# Autodesk Inventor assembly: PC104 Stack Ultra Low Profile
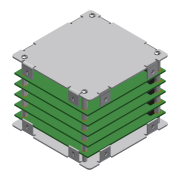
[picture p0: Inventor's stored thumbnail of the model, 180x180]
Saved by Autodesk Inventor 2018 (Build 220112000, 112)
## iProperties
Created: 2018-12-12
Part Number: PC104 Stack Ultra Low Profile
Document SubType Name: Assembly
Designer: R.P.SMITH
Mass: 216.229 g
Surface Area: 1807.71 cm^2
Volume: 132.857 cm^3
Density: 1.62753 g/cm^3
Author: R.P.SMITH
## Documents named in this file (10)
- D:\Documents\College\Semesters\4 - Fall\Senior Project 2\CADD Files\PC104 STACK ULTRA LOW PROFILE.iam
- D:\Documents\College\Semesters\4 - Fall\Senior Project 2\CADD Files\McMaster\93505A925_ALUM MALE-FEM THRDED HEX STANDOFF.ipt
- D:\Documents\College\Semesters\4 - Fall\Senior Project 2\CADD Files\Custom Parts\END MOUNT PC104 TOP.iam
- D:\Documents\College\Semesters\4 - Fall\Senior Project 2\CADD Files\McMaster\91772A106_18-8 SS PAN HEAD PHILLIPS MACHINE SCREW.ipt
- D:\Documents\College\Semesters\4 - Fall\Senior Project 2\CADD Files\Custom Parts\END MOUNT PC104 BOTTOM.iam
- D:\Documents\College\Semesters\4 - Fall\Senior Project 2\CADD Files\PC104 ISA BOARD VERY LOW PROFILE.iam
- D:\Documents\College\Semesters\4 - Fall\Senior Project 2\CADD Files\McMaster\93505A102_ALUM MALE-FEM THRDED HEX STANDOFF.ipt
- D:\Documents\College\Semesters\4 - Fall\Senior Project 2\CADD Files\McMaster\92510A696_ALUM UNTHRD SPACER.ipt
- D:\Documents\College\Semesters\4 - Fall\Senior Project 2\CADD Files\McMaster\91780A529_ALUM FEM THRDED HEX STANDOFF.ipt
- D:\Documents\College\Semesters\4 - Fall\Senior Project 2\CADD Files\McMaster\91772A112_18-8 SS PAN HEAD PHILLIPS MACHINE SCREW.ipt
## Components (39 placed, 9 different names)
1. 91772A106_18-8 SS PAN HEAD PHILLIPS MACHINE SCREW:1 — Insert:33
2. 91772A106_18-8 SS PAN HEAD PHILLIPS MACHINE SCREW:2 — Insert:34
3. 91772A106_18-8 SS PAN HEAD PHILLIPS MACHINE SCREW:3 — Insert:32
4. 91772A106_18-8 SS PAN HEAD PHILLIPS MACHINE SCREW:4 — Insert:31
5. END MOUNT PC104 TOP:2 [sub-assembly] — Insert:31, Insert:32, Insert:33, Insert:34, Insert:35, Insert:36, Insert:37, Insert:38
6. 93505A925_ALUM MALE-FEM THRDED HEX STANDOFF:1 — Insert:35, Insert:40
7. 93505A925_ALUM MALE-FEM THRDED HEX STANDOFF:2 — Insert:36
8. 93505A925_ALUM MALE-FEM THRDED HEX STANDOFF:3 — Insert:38, Insert:39
9. 93505A925_ALUM MALE-FEM THRDED HEX STANDOFF:4 — Insert:37
10. PC104 ISA BOARD VERY LOW PROFILE:4 [sub-assembly] — Insert:39, Insert:40, Mate:16, Insert:41, Insert:42, Insert:43, Insert:44
11. 93505A102_ALUM MALE-FEM THRDED HEX STANDOFF:1 — Insert:41
12. 93505A102_ALUM MALE-FEM THRDED HEX STANDOFF:2 — Insert:42
13. 93505A102_ALUM MALE-FEM THRDED HEX STANDOFF:3 — Insert:43
14. 93505A102_ALUM MALE-FEM THRDED HEX STANDOFF:4 — Insert:44
15. PC104 ISA BOARD VERY LOW PROFILE:3 [sub-assembly] — Mate:16, Mate:17, Insert:45, Insert:46, Insert:47, Insert:48
16. 93505A102_ALUM MALE-FEM THRDED HEX STANDOFF:5 — Insert:48
17. 93505A102_ALUM MALE-FEM THRDED HEX STANDOFF:12 — Insert:46
18. 93505A102_ALUM MALE-FEM THRDED HEX STANDOFF:14 — Insert:47
19. 93505A102_ALUM MALE-FEM THRDED HEX STANDOFF:13 — Insert:45
20. PC104 ISA BOARD VERY LOW PROFILE:2 [sub-assembly] — Mate:17, Mate:18, Insert:49, Insert:50, Insert:51, Insert:52
21. 93505A102_ALUM MALE-FEM THRDED HEX STANDOFF:6 — Insert:52
22. 93505A102_ALUM MALE-FEM THRDED HEX STANDOFF:9 — Insert:50
23. 93505A102_ALUM MALE-FEM THRDED HEX STANDOFF:10 — Insert:49
24. 93505A102_ALUM MALE-FEM THRDED HEX STANDOFF:11 — Insert:51
25. PC104 ISA BOARD VERY LOW PROFILE:1 [sub-assembly] — Mate:18, Mate:19, Insert:63, Insert:64, Insert:65, Insert:66
26. 91780A529_ALUM FEM THRDED HEX STANDOFF:1 — Insert:63
27. 91780A529_ALUM FEM THRDED HEX STANDOFF:2 — Insert:64
28. 91780A529_ALUM FEM THRDED HEX STANDOFF:3 — Insert:65
29. 91780A529_ALUM FEM THRDED HEX STANDOFF:4 — Insert:66
30. PC104 ISA BOARD VERY LOW PROFILE:5 [sub-assembly] — Mate:19, Mate:20, Insert:57, Insert:59, Insert:61, Insert:62
31. 92510A696_ALUM UNTHRD SPACER:1 — Insert:62
32. 92510A696_ALUM UNTHRD SPACER:2 — Insert:57, Insert:58
33. 92510A696_ALUM UNTHRD SPACER:3 — Insert:61
34. 92510A696_ALUM UNTHRD SPACER:4 — Insert:59, Insert:60
35. END MOUNT PC104 BOTTOM:1 [sub-assembly] — Mate:20, Insert:58, Insert:60, Insert:67, Insert:68, Insert:69, Insert:70
36. 91772A112_18-8 SS PAN HEAD PHILLIPS MACHINE SCREW:1 — Insert:67
37. 91772A112_18-8 SS PAN HEAD PHILLIPS MACHINE SCREW:2 — Insert:68
38. 91772A112_18-8 SS PAN HEAD PHILLIPS MACHINE SCREW:3 — Insert:70
39. 91772A112_18-8 SS PAN HEAD PHILLIPS MACHINE SCREW:4 — Insert:69
## Relationships (49: Insert 36, Mate 13)
- [Mate]: PC104 ISA BOARD VERY LOW PROFILE:2 ↔ PC104 ISA BOARD VERY LOW PROFILE:1
- [Mate]: PC104 ISA BOARD VERY LOW PROFILE:2 ↔ PC104 ISA BOARD VERY LOW PROFILE:1
- [Mate]: PC104 ISA BOARD VERY LOW PROFILE:3 ↔ PC104 ISA BOARD VERY LOW PROFILE:2
- [Mate]: PC104 ISA BOARD VERY LOW PROFILE:3 ↔ PC104 ISA BOARD VERY LOW PROFILE:2
- [Mate]: PC104 ISA BOARD VERY LOW PROFILE:4 ↔ PC104 ISA BOARD VERY LOW PROFILE:3
- [Mate]: PC104 ISA BOARD VERY LOW PROFILE:4 ↔ PC104 ISA BOARD VERY LOW PROFILE:3
- [Mate]: PC104 ISA BOARD VERY LOW PROFILE:1 ↔ PC104 ISA BOARD VERY LOW PROFILE:5
- [Mate]: PC104 ISA BOARD VERY LOW PROFILE:1 ↔ PC104 ISA BOARD VERY LOW PROFILE:5
- Insert:31: 91772A106_18-8 SS PAN HEAD PHILLIPS MACHINE SCREW:4 ↔ END MOUNT PC104 TOP:2
- Insert:32: 91772A106_18-8 SS PAN HEAD PHILLIPS MACHINE SCREW:3 ↔ END MOUNT PC104 TOP:2
- Insert:33: 91772A106_18-8 SS PAN HEAD PHILLIPS MACHINE SCREW:1 ↔ END MOUNT PC104 TOP:2
- Insert:34: 91772A106_18-8 SS PAN HEAD PHILLIPS MACHINE SCREW:2 ↔ END MOUNT PC104 TOP:2
- Insert:35: END MOUNT PC104 TOP:2 ↔ 93505A925_ALUM MALE-FEM THRDED HEX STANDOFF:1
- Insert:36: END MOUNT PC104 TOP:2 ↔ 93505A925_ALUM MALE-FEM THRDED HEX STANDOFF:2
- Insert:37: END MOUNT PC104 TOP:2 ↔ 93505A925_ALUM MALE-FEM THRDED HEX STANDOFF:4
- Insert:38: END MOUNT PC104 TOP:2 ↔ 93505A925_ALUM MALE-FEM THRDED HEX STANDOFF:3
- Insert:39: 93505A925_ALUM MALE-FEM THRDED HEX STANDOFF:3 ↔ PC104 ISA BOARD VERY LOW PROFILE:4
- Insert:40: 93505A925_ALUM MALE-FEM THRDED HEX STANDOFF:1 ↔ PC104 ISA BOARD VERY LOW PROFILE:4
- Mate:16 (9.525 mm): PC104 ISA BOARD VERY LOW PROFILE:4 ↔ PC104 ISA BOARD VERY LOW PROFILE:3
- Mate:17 (9.525 mm): PC104 ISA BOARD VERY LOW PROFILE:3 ↔ PC104 ISA BOARD VERY LOW PROFILE:2
- Mate:18 (9.525 mm): PC104 ISA BOARD VERY LOW PROFILE:2 ↔ PC104 ISA BOARD VERY LOW PROFILE:1
- Mate:19 (9.525 mm): PC104 ISA BOARD VERY LOW PROFILE:1 ↔ PC104 ISA BOARD VERY LOW PROFILE:5
- Insert:41: PC104 ISA BOARD VERY LOW PROFILE:4 ↔ 93505A102_ALUM MALE-FEM THRDED HEX STANDOFF:1
- Insert:42: PC104 ISA BOARD VERY LOW PROFILE:4 ↔ 93505A102_ALUM MALE-FEM THRDED HEX STANDOFF:2
- Insert:43: PC104 ISA BOARD VERY LOW PROFILE:4 ↔ 93505A102_ALUM MALE-FEM THRDED HEX STANDOFF:3
- Insert:44: PC104 ISA BOARD VERY LOW PROFILE:4 ↔ 93505A102_ALUM MALE-FEM THRDED HEX STANDOFF:4
- Insert:45: PC104 ISA BOARD VERY LOW PROFILE:3 ↔ 93505A102_ALUM MALE-FEM THRDED HEX STANDOFF:13
- Insert:46: PC104 ISA BOARD VERY LOW PROFILE:3 ↔ 93505A102_ALUM MALE-FEM THRDED HEX STANDOFF:12
- Insert:47: PC104 ISA BOARD VERY LOW PROFILE:3 ↔ 93505A102_ALUM MALE-FEM THRDED HEX STANDOFF:14
- Insert:48: PC104 ISA BOARD VERY LOW PROFILE:3 ↔ 93505A102_ALUM MALE-FEM THRDED HEX STANDOFF:5
- Insert:49: PC104 ISA BOARD VERY LOW PROFILE:2 ↔ 93505A102_ALUM MALE-FEM THRDED HEX STANDOFF:10
- Insert:50: PC104 ISA BOARD VERY LOW PROFILE:2 ↔ 93505A102_ALUM MALE-FEM THRDED HEX STANDOFF:9
- Insert:51: PC104 ISA BOARD VERY LOW PROFILE:2 ↔ 93505A102_ALUM MALE-FEM THRDED HEX STANDOFF:11
- Insert:52: PC104 ISA BOARD VERY LOW PROFILE:2 ↔ 93505A102_ALUM MALE-FEM THRDED HEX STANDOFF:6
- Mate:20 (9.525 mm): PC104 ISA BOARD VERY LOW PROFILE:5 ↔ END MOUNT PC104 BOTTOM:1
- Insert:57: PC104 ISA BOARD VERY LOW PROFILE:5 ↔ 92510A696_ALUM UNTHRD SPACER:2
- Insert:58: 92510A696_ALUM UNTHRD SPACER:2 ↔ END MOUNT PC104 BOTTOM:1
- Insert:59: PC104 ISA BOARD VERY LOW PROFILE:5 ↔ 92510A696_ALUM UNTHRD SPACER:4
- Insert:60: 92510A696_ALUM UNTHRD SPACER:4 ↔ END MOUNT PC104 BOTTOM:1
- Insert:61: PC104 ISA BOARD VERY LOW PROFILE:5 ↔ 92510A696_ALUM UNTHRD SPACER:3
- Insert:62: PC104 ISA BOARD VERY LOW PROFILE:5 ↔ 92510A696_ALUM UNTHRD SPACER:1
- Insert:63: PC104 ISA BOARD VERY LOW PROFILE:1 ↔ 91780A529_ALUM FEM THRDED HEX STANDOFF:1
- Insert:64: PC104 ISA BOARD VERY LOW PROFILE:1 ↔ 91780A529_ALUM FEM THRDED HEX STANDOFF:2
- Insert:65: PC104 ISA BOARD VERY LOW PROFILE:1 ↔ 91780A529_ALUM FEM THRDED HEX STANDOFF:3
- Insert:66: PC104 ISA BOARD VERY LOW PROFILE:1 ↔ 91780A529_ALUM FEM THRDED HEX STANDOFF:4
- Insert:67: END MOUNT PC104 BOTTOM:1 ↔ 91772A112_18-8 SS PAN HEAD PHILLIPS MACHINE SCREW:1
- Insert:68: END MOUNT PC104 BOTTOM:1 ↔ 91772A112_18-8 SS PAN HEAD PHILLIPS MACHINE SCREW:2
- Insert:69: END MOUNT PC104 BOTTOM:1 ↔ 91772A112_18-8 SS PAN HEAD PHILLIPS MACHINE SCREW:4
- Insert:70: END MOUNT PC104 BOTTOM:1 ↔ 91772A112_18-8 SS PAN HEAD PHILLIPS MACHINE SCREW:3
